# Autodesk Inventor assembly: Operator Junction Box Assembly
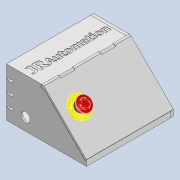
[picture p0: Inventor's stored thumbnail of the model, 180x180]
Saved by Autodesk Inventor 2022 (Build 260153000, 153)
## iProperties
Created: 2022-01-10
Part Number: Operator Junction Box Assembly
Document SubType Name: Assembly
Designer: Coy
Author: Coy
## Documents named in this file (6)
- H:\3D Files\Project 3D Models\Breakfast Maker 2000\Assemblys\Operator Junction Box Assembly.iam
- H:\3D Files\Project 3D Models\Breakfast Maker 2000\3D Printed Parts\Operator Junction Box Main.ipt
- H:\3D Files\Project 3D Models\Breakfast Maker 2000\Sensors\e-stop-switch\e_stop_switch_asm.iam
- H:\3D Files\Project 3D Models\Breakfast Maker 2000\Thread Inserts\M5 7mm OD 6mm Deep Threaded Insert.ipt
- H:\3D Files\Project 3D Models\Breakfast Maker 2000\3D Printed Parts\Operator Junction Box Side Panel.ipt
- H:\3D Files\Project 3D Models\Breakfast Maker 2000\Nuts and Bolts\M5 x 8 Socket Head Bolt.ipt
## Components (11 placed, 5 different names)
1. Operator Junction Box Main:1 — Mate:1, Mate:2, Mate:3, Mate:4, Mate:5, Mate:6, Mate:7, Mate:10
2. e_stop_switch_asm:1 [sub-assembly] — Mate:1, Mate:2
3. M5 7mm OD 6mm Deep Threaded Insert:1 — Mate:3, Flush:1, Flush:2, Flush:3, Mate:7
4. M5 7mm OD 6mm Deep Threaded Insert:2 — Mate:4, Flush:2, Mate:8
5. M5 7mm OD 6mm Deep Threaded Insert:3 — Mate:6, Flush:1
6. M5 7mm OD 6mm Deep Threaded Insert:4 — Mate:5, Flush:3, Mate:9
7. Operator Junction Box Side Panel:1 — Mate:8, Mate:9, Mate:10, Mate:11, Mate:12, Mate:13, Mate:14, Mate:15
8. M5 x 8 Socket Head Bolt:1 — Mate:11, Flush:6
9. M5 x 8 Socket Head Bolt:2 — Mate:12, Flush:5
10. M5 x 8 Socket Head Bolt:3 — Mate:14, Flush:4
11. M5 x 8 Socket Head Bolt:4 — Mate:13, Flush:4, Flush:5, Flush:6, Mate:15
## Relationships (21: Mate 15, Flush 6)
- Mate:1: Operator Junction Box Main:1 ↔ e_stop_switch_asm:1
- Mate:2: Operator Junction Box Main:1 ↔ e_stop_switch_asm:1
- Mate:3: Operator Junction Box Main:1 ↔ M5 7mm OD 6mm Deep Threaded Insert:1
- Mate:4: Operator Junction Box Main:1 ↔ M5 7mm OD 6mm Deep Threaded Insert:2
- Mate:5: Operator Junction Box Main:1 ↔ M5 7mm OD 6mm Deep Threaded Insert:4
- Mate:6: Operator Junction Box Main:1 ↔ M5 7mm OD 6mm Deep Threaded Insert:3
- Flush:1: M5 7mm OD 6mm Deep Threaded Insert:1 ↔ M5 7mm OD 6mm Deep Threaded Insert:3
- Flush:2: M5 7mm OD 6mm Deep Threaded Insert:1 ↔ M5 7mm OD 6mm Deep Threaded Insert:2
- Flush:3: M5 7mm OD 6mm Deep Threaded Insert:1 ↔ M5 7mm OD 6mm Deep Threaded Insert:4
- Mate:7: Operator Junction Box Main:1 ↔ M5 7mm OD 6mm Deep Threaded Insert:1
- Mate:8: M5 7mm OD 6mm Deep Threaded Insert:2 ↔ Operator Junction Box Side Panel:1
- Mate:9: M5 7mm OD 6mm Deep Threaded Insert:4 ↔ Operator Junction Box Side Panel:1
- Mate:10 (0.05 mm): Operator Junction Box Main:1 ↔ Operator Junction Box Side Panel:1
- Mate:11: Operator Junction Box Side Panel:1 ↔ M5 x 8 Socket Head Bolt:1
- Mate:12: Operator Junction Box Side Panel:1 ↔ M5 x 8 Socket Head Bolt:2
- Mate:13: Operator Junction Box Side Panel:1 ↔ M5 x 8 Socket Head Bolt:4
- Mate:14: Operator Junction Box Side Panel:1 ↔ M5 x 8 Socket Head Bolt:3
- Flush:4: M5 x 8 Socket Head Bolt:3 ↔ M5 x 8 Socket Head Bolt:4
- Flush:5: M5 x 8 Socket Head Bolt:2 ↔ M5 x 8 Socket Head Bolt:4
- Flush:6: M5 x 8 Socket Head Bolt:1 ↔ M5 x 8 Socket Head Bolt:4
- Mate:15: Operator Junction Box Side Panel:1 ↔ M5 x 8 Socket Head Bolt:4
